# Autodesk Inventor assembly: bett_V2_elem
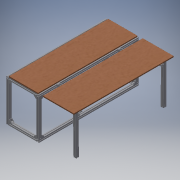
[picture p0: Inventor's stored thumbnail of the model, 180x180]
Saved by Autodesk Inventor 2018 (Build 220112000, 112)
## iProperties
Created: 2020-04-19
Part Number: bett_V2_elem
Material: Generisch
Document SubType Name: Assembly
Designer: wepet
Author: wepet
## Documents named in this file (5)
- C:\Users\wepet\Downloads\anhaenger\current\details\bett\bett_V2\bett_V2.iam
- C:\Users\wepet\Downloads\anhaenger\current\details\bett\bett_V2\bett_V2_teil4_bein.iam
- C:\Users\wepet\Downloads\anhaenger\current\details\bett\bett_V2\bett_V2_teil2_deckplatte.ipt
- C:\Users\wepet\Downloads\anhaenger\current\details\bett\bett_V2\bett_V2_teil3_klappe.iam
- C:\Users\wepet\Downloads\anhaenger\current\details\bett\bett_V2\bett_V2_teil1_sitzbank.iam
## Components (5 placed, 4 different names)
1. bett_V2_teil2_deckplatte:1 — Fluchtend:1, Drehbar:2
2. bett_V2_teil3_klappe:1 [sub-assembly] — Drehbar:1, Drehbar:3, Drehbar:4
3. bett_V2_teil1_sitzbank:1 [sub-assembly] — Passend:1, Passend:2, Passend:3, Drehbar:1, Fluchtend:1, Drehbar:2
4. bett_V2_teil4_bein:1 [sub-assembly] — Drehbar:3
5. bett_V2_teil4_bein:2 [sub-assembly] — Drehbar:4
## Relationships (8: RevoluteJoint 4, Mate 3, Flush 1)
- Passend:1 [Mate]: bett_V2_teil1_sitzbank:1
- Passend:2 [Mate]: bett_V2_teil1_sitzbank:1
- Passend:3 [Mate]: bett_V2_teil1_sitzbank:1
- Drehbar:1 [RevoluteJoint]: bett_V2_teil3_klappe:1 ↔ bett_V2_teil1_sitzbank:1
- Fluchtend:1 [Flush]: bett_V2_teil2_deckplatte:1 ↔ bett_V2_teil1_sitzbank:1
- Drehbar:2 [RevoluteJoint]: bett_V2_teil2_deckplatte:1 ↔ bett_V2_teil1_sitzbank:1
- Drehbar:3 [RevoluteJoint]: bett_V2_teil3_klappe:1 ↔ bett_V2_teil4_bein:1
- Drehbar:4 [RevoluteJoint]: bett_V2_teil3_klappe:1 ↔ bett_V2_teil4_bein:2
